# Autodesk Inventor assembly: Сборка2
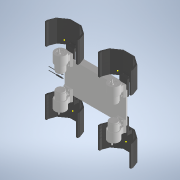
[picture p0: Inventor's stored thumbnail of the model, 180x180]
Saved by Autodesk Inventor 2022 (Build 260153000, 153)
## iProperties
Created: 2023-05-17
Part Number: Сборка2
Document SubType Name: Assembly
Designer: korsh624
Author: korsh624
## Documents named in this file (8)
- C:\git\robot_01\design\Сборка2.iam
- C:\git\robot_01\design\драйвер.ipt
- C:\git\robot_01\design\Receiver.ipt
- C:\git\robot_01\design\MEGA 2560 PRO (EMBED).iam
- C:\git\robot_01\design\2 Relay Module v2.ipt
- C:\git\robot_01\design\корпус.ipt
- C:\git\robot_01\design\motor_krilo.iam
- C:\git\robot_01\design\base.ipt
## Components (11 placed, 7 different names)
1. драйвер:1 — Заподлицо:1, Заподлицо:3, Заподлицо:5, Совмещение:1, Заподлицо:6, Заподлицо:8, Совмещение:2
2. драйвер:2 — Заподлицо:1, Совмещение:1, Заподлицо:6, Заподлицо:7, Заподлицо:10
3. Receiver:1 — Заподлицо:4, Заподлицо:8, Заподлицо:9
4. MEGA 2560 PRO (EMBED):1 [sub-assembly] — Заподлицо:5, Совмещение:2, Совмещение:3, Заподлицо:10
5. 2 Relay Module v2:1 — Заподлицо:3, Заподлицо:4, Заподлицо:7, Заподлицо:9, Совмещение:3, Заподлицо:11
6. корпус:1 — Заподлицо:11, Заподлицо:18, Заподлицо:19
7. motor_krilo:1 [sub-assembly] — Заподлицо:12, Заподлицо:13, Совмещение:4, Заподлицо:16, Совмещение:6, Заподлицо:18
8. motor_krilo:2 [sub-assembly] — Заподлицо:12, Заподлицо:13, Совмещение:4, Заподлицо:17, Заподлицо:19, Заподлицо:20
9. motor_krilo:3 [sub-assembly] — Заподлицо:14, Заподлицо:15, Совмещение:5, Заподлицо:16, Заподлицо:17
10. motor_krilo:4 [sub-assembly] — Заподлицо:14, Заподлицо:15, Совмещение:5, Совмещение:6
11. base:1 — Заподлицо:20
## Relationships (25: Flush 19, Mate 6)
- Заподлицо:1 [Flush]: драйвер:1 ↔ драйвер:2
- Заподлицо:3 [Flush]: драйвер:1 ↔ 2 Relay Module v2:1
- Заподлицо:4 [Flush]: Receiver:1 ↔ 2 Relay Module v2:1
- Заподлицо:5 [Flush]: драйвер:1 ↔ MEGA 2560 PRO (EMBED):1
- Совмещение:1 [Mate] (5 mm): драйвер:1 ↔ драйвер:2
- Заподлицо:6 [Flush]: драйвер:1 ↔ драйвер:2
- Заподлицо:7 [Flush]: драйвер:2 ↔ 2 Relay Module v2:1
- Заподлицо:8 [Flush]: драйвер:1 ↔ Receiver:1
- Заподлицо:9 [Flush]: Receiver:1 ↔ 2 Relay Module v2:1
- Совмещение:2 [Mate] (5 mm): драйвер:1 ↔ MEGA 2560 PRO (EMBED):1
- Совмещение:3 [Mate] (5 mm): MEGA 2560 PRO (EMBED):1 ↔ 2 Relay Module v2:1
- Заподлицо:10 [Flush]: драйвер:2 ↔ MEGA 2560 PRO (EMBED):1
- Заподлицо:11 [Flush]: 2 Relay Module v2:1 ↔ корпус:1
- Заподлицо:12 [Flush]: motor_krilo:1 ↔ motor_krilo:2
- Заподлицо:13 [Flush]: motor_krilo:1 ↔ motor_krilo:2
- Заподлицо:14 [Flush]: motor_krilo:3 ↔ motor_krilo:4
- Заподлицо:15 [Flush]: motor_krilo:3 ↔ motor_krilo:4
- Совмещение:4 [Mate] (200 mm): motor_krilo:1 ↔ motor_krilo:2
- Совмещение:5 [Mate] (200 mm): motor_krilo:3 ↔ motor_krilo:4
- Заподлицо:16 [Flush]: motor_krilo:1 ↔ motor_krilo:3
- Совмещение:6 [Mate] (80 mm): motor_krilo:1 ↔ motor_krilo:4
- Заподлицо:17 [Flush]: motor_krilo:2 ↔ motor_krilo:3
- Заподлицо:18 [Flush]: корпус:1 ↔ motor_krilo:1
- Заподлицо:19 [Flush] (40 mm): корпус:1 ↔ motor_krilo:2
- Заподлицо:20 [Flush]: motor_krilo:2 ↔ base:1
